# Autodesk Inventor assembly: Piston rod
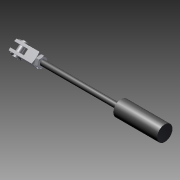
[picture p0: Inventor's stored thumbnail of the model, 180x180]
Saved by Autodesk Inventor 2012 (Build 160160000, 160)
## iProperties
Created: 2013-01-17
Part Number: Piston rod
Document SubType Name: Assembly
Designer: William
Author: William
## Documents named in this file (6)
- Z:\UserData\Documents\Inventor\team1885frc\Robot2013\Launcher\Piston\Piston rod.iam
- Z:\UserData\Documents\Inventor\team1885frc\Robot2013\Launcher\Piston\.75 inch\0430_rod.ipt
- Z:\UserData\Documents\Inventor\team1885frc\Robot2013\Launcher\Piston\.75 inch\D-14055.ipt
- Z:\UserData\Documents\Inventor\team1885frc\Robot2013\Launcher\Piston\.75 inch\D-8381.ipt
- Z:\UserData\Documents\Inventor\team1885frc\Robot2013\Launcher\Piston\.75 inch\D-5866.ipt
- Z:\UserData\Documents\Inventor\team1885frc\Robot2013\Launcher\Piston\.75 inch\D-344.ipt
## Components (6 placed, 5 different names)
1. 0430_rod:1 — Mate:9, Flush:1
2. D-14055:1 — Mate:1, Mate:4, Mate:5, Mate:7, Mate:8, Angle:1
3. D-8381:1 — Mate:1, Mate:2, Mate:3, Mate:6
4. D-5866:1 — Mate:2, Mate:3, Mate:4
5. D-5866:2 — Mate:5, Mate:6
6. D-344:1 — Mate:7, Mate:8, Angle:1, Mate:9, Flush:1
## Relationships (11: Mate 9, Angle 1, Flush 1)
- Mate:1: D-14055:1 ↔ D-8381:1
- Mate:2: D-8381:1 ↔ D-5866:1
- Mate:3: D-8381:1 ↔ D-5866:1
- Mate:4: D-14055:1 ↔ D-5866:1
- Mate:5: D-14055:1 ↔ D-5866:2
- Mate:6: D-8381:1 ↔ D-5866:2
- Mate:7: D-14055:1 ↔ D-344:1
- Mate:8: D-14055:1 ↔ D-344:1
- Angle:1 (0 deg): D-14055:1 ↔ D-344:1
- Mate:9: 0430_rod:1 ↔ D-344:1
- Flush:1: 0430_rod:1 ↔ D-344:1
